# Autodesk Inventor assembly: y-carriage
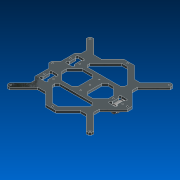
[picture p0: Inventor's stored thumbnail of the model, 180x180]
Saved by Autodesk Inventor 2021 (Build 250183000, 183)
## iProperties
Created: 2021-03-09
Part Number: y-carriage
Document SubType Name: Assembly
Designer: Alex
Author: Alex
## Documents named in this file (5)
- C:\Users\Alex\Documents\PrusaMini\V1\IPT\ASSEMBLY\y-carriage.iam
- C:\Users\Alex\Documents\PrusaMini\V1\IPT\PARTS\y-carriage.ipt
- MINI-y-carriage.ipt
- C:\Users\Alex\Documents\PrusaMini\V1\IPT\PARTS\bearing-clip.ipt
- C:\Users\Alex\Documents\PrusaMini\V1\IPT\PARTS\lm8uu.ipt
## Components (3 placed, 3 different names)
1. MINI-y-carriage:1 — Tangent:1, Tangent:2, Mate:1, Flush:1
2. bearing-clip:1 — Tangent:1, Tangent:2, Mate:1, Flush:1, Tangent:3, Tangent:4, Flush:2
3. lm8uu:1 — Tangent:3, Tangent:4, Flush:2
## Relationships (7: Tangent 4, Flush 2, Mate 1)
- Tangent:1: MINI-y-carriage:1 ↔ bearing-clip:1
- Tangent:2: MINI-y-carriage:1 ↔ bearing-clip:1
- Mate:1: MINI-y-carriage:1 ↔ bearing-clip:1
- Flush:1 (-2.5 mm): MINI-y-carriage:1 ↔ bearing-clip:1
- Tangent:3: bearing-clip:1 ↔ lm8uu:1
- Tangent:4: bearing-clip:1 ↔ lm8uu:1
- Flush:2 (3 mm): bearing-clip:1 ↔ lm8uu:1
